# Autodesk Inventor assembly: neveRest with 15T pinion_MIR1
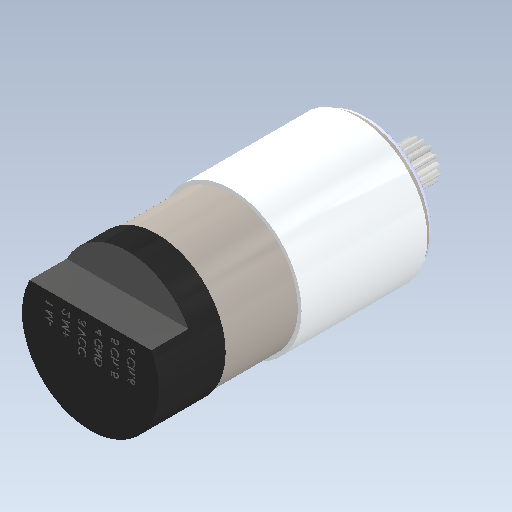
[picture p0: Inventor's stored thumbnail of the model, 512x512]
Saved by Autodesk Inventor 2020.2 (Build 242310000, 310)
## iProperties
Created: 2020-02-27
Part Number: neveRest with 15T pinion_MIR1
Document SubType Name: Assembly
Designer: deli
Author: deli
## Documents named in this file (3)
- C:\Users\deli\OneDrive - Eastside Preparatory School\FTC\Chassi\neveRest with 15T pinion_MIR1.iam
- C:\Users\deli\OneDrive - Eastside Preparatory School\FTC\Chassi\am-3104 NeveRest Motor_MIR1.ipt
- C:\Users\deli\OneDrive - Eastside Preparatory School\FTC\Chassi\15T+pinion+3.2mm+bore+motor - Copy_MIR1.ipt
## Components (2 placed, 2 different names)
1. am-3104 NeveRest Motor_MIR1:1 — Mate:2, Mate:1
2. 15T+pinion+3.2mm+bore+motor - Copy_MIR1:1 — Mate:2, Mate:1
## Relationships (2: Mate 2)
- Mate:2 (0.7874 mm): am-3104 NeveRest Motor_MIR1:1 ↔ 15T+pinion+3.2mm+bore+motor - Copy_MIR1:1
- Mate:1: am-3104 NeveRest Motor_MIR1:1 ↔ 15T+pinion+3.2mm+bore+motor - Copy_MIR1:1
